# Autodesk Inventor assembly: GearBox Assembly_MIR_MIR
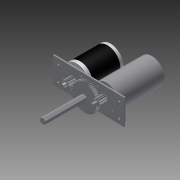
[picture p0: Inventor's stored thumbnail of the model, 180x180]
Saved by Autodesk Inventor 2015 (Build 190159000, 159)
## iProperties
Created: 2015-01-14
Part Number: GearBox Assembly_MIR_MIR
Document SubType Name: Assembly
Designer: chapale16
Author: whitaus15
## Documents named in this file (7)
- \\LHSSVR02\Homedirs\Robotics Club\CAD Model 2015\GearBox Assembly_MIR_MIR.iam
- \\LHSSVR02\Homedirs\Robotics Club\CAD Model 2015\Imported Components\2014-DiaD-Mecanum\217-3107-001_KEY_MIR_MIR.ipt
- \\LHSSVR02\Homedirs\Robotics Club\CAD Model 2015\Imported Components\2014-DiaD-Mecanum\Mecanum Axle_MIR_MIR.ipt
- \\LHSSVR02\Homedirs\Robotics Club\CAD Model 2015\Imported Components\2014-DiaD-Mecanum\217-2000 - CIM Motor_MIR_MIR.ipt
- \\LHSSVR02\Homedirs\Robotics Club\CAD Model 2015\Parts Folder\Gear Boxes\Imported Components\Toughbox-mini\Toughbox-mini_d02_MIR4_MIR.ipt
- \\LHSSVR02\Homedirs\Robotics Club\CAD Model 2015\Parts Folder\Gear Boxes\Imported Components\Toughbox-mini\Toughbox_d06_MIR3_MIR_MIR.ipt
- \\LHSSVR02\Homedirs\Robotics Club\CAD Model 2015\Parts Folder\Motors\Imported Components\MOT_MiniCIMMotor_217-3371.ipt\MOT_MiniCIMMotor_217-3371.ipt_MIR_MIR.ipt
## Components (7 placed, 6 different names)
1. 217-3107-001_KEY_MIR_MIR:1 — Insert:1
2. Mecanum Axle_MIR_MIR:1 — Flush:1, Mate:4, Mate:1, Mate:2, Mate:3
3. 217-2000 - CIM Motor_MIR_MIR:1 — Insert:1, Insert:2
4. Toughbox-mini_d02_MIR4_MIR:1 — Flush:1, Insert:2, Mate:4, Mate:5, Mate:6
5. Toughbox_d06_MIR3_MIR_MIR:1 — Mate:1, Mate:2, Mate:3
6. MOT_MiniCIMMotor_217-3371.ipt_MIR_MIR:1 — Mate:5, Mate:7, Mate:6
7. 217-3107-001_KEY_MIR_MIR:2 — Mate:7
## Relationships (10: Mate 7, Insert 2, Flush 1)
- Insert:1 (1.27 mm): 217-3107-001_KEY_MIR_MIR:1 ↔ 217-2000 - CIM Motor_MIR_MIR:1
- Flush:1: Mecanum Axle_MIR_MIR:1 ↔ Toughbox-mini_d02_MIR4_MIR:1
- Insert:2: 217-2000 - CIM Motor_MIR_MIR:1 ↔ Toughbox-mini_d02_MIR4_MIR:1
- Mate:4: Mecanum Axle_MIR_MIR:1 ↔ Toughbox-mini_d02_MIR4_MIR:1
- Mate:1: Mecanum Axle_MIR_MIR:1 ↔ Toughbox_d06_MIR3_MIR_MIR:1
- Mate:2: Mecanum Axle_MIR_MIR:1 ↔ Toughbox_d06_MIR3_MIR_MIR:1
- Mate:3: Mecanum Axle_MIR_MIR:1 ↔ Toughbox_d06_MIR3_MIR_MIR:1
- Mate:5: Toughbox-mini_d02_MIR4_MIR:1 ↔ MOT_MiniCIMMotor_217-3371.ipt_MIR_MIR:1
- Mate:7: MOT_MiniCIMMotor_217-3371.ipt_MIR_MIR:1 ↔ 217-3107-001_KEY_MIR_MIR:2
- Mate:6: Toughbox-mini_d02_MIR4_MIR:1 ↔ MOT_MiniCIMMotor_217-3371.ipt_MIR_MIR:1
